# Autodesk Inventor assembly: Zmotionassembly(right)1
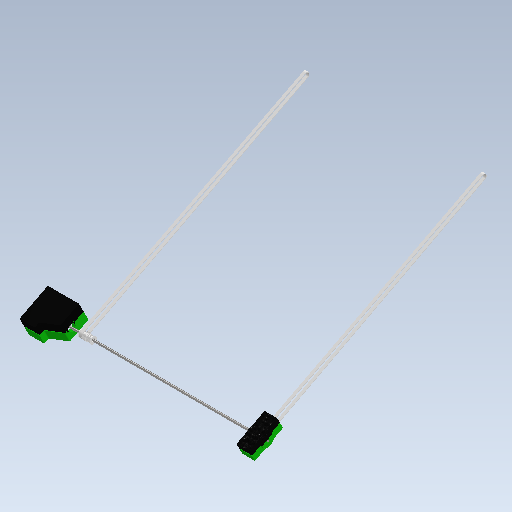
[picture p0: Inventor's stored thumbnail of the model, 512x512]
Saved by Autodesk Inventor 2020.4 (Build 244396000, 396)
## iProperties
Created: 2021-03-29
Part Number: Zmotionassembly(right)1
Document SubType Name: Assembly
Designer: AOB
Mass: 162.106 g
Surface Area: 1029.45 cm^2
Volume: 151.649 cm^3
Density: 1.06896 g/cm^3
Author: AOB
## Documents named in this file (5)
- C:\Users\marti\Documents\Inventor\ProjectBoron\Boron Ultima\Zmotionassembly(right)1.iam
- C:\Users\marti\Documents\Inventor\ProjectBoron\Boron Ultima\Z-powertrain(right)1.iam
- C:\Users\marti\Documents\Inventor\ProjectBoron\Boron Ultima\bottom idler housing(right)1.iam
- C:\Users\marti\Documents\Inventor\ProjectBoron\Boron Ultima\zmotorblock(right)1.iam
- C:\Users\marti\Documents\Inventor\ProjectBoron\Boron Ultima\z-belt(right)1.ipt
## Components (5 placed, 4 different names)
1. Z-powertrain(right)1:1 [sub-assembly] — Flush:1, Mate:2, Flush:2, Mate:3, Rotational:2, Rotational:3
2. bottom idler housing(right)1:1 [sub-assembly] — Flush:1, Mate:2, Angle:1
3. zmotorblock(right)1:1 [sub-assembly] — Flush:2, Mate:3, Angle:2
4. z-belt(right)1:1 — Angle:1, Angle:3, Rotational:2
5. z-belt(right)1:2 — Angle:3, Angle:2, Rotational:3
## Relationships (9: Angle 3, Flush 2, Mate 2, RevoluteJoint 2)
- Flush:1: Z-powertrain(right)1:1 ↔ bottom idler housing(right)1:1
- Mate:2: Z-powertrain(right)1:1 ↔ bottom idler housing(right)1:1
- Flush:2: Z-powertrain(right)1:1 ↔ zmotorblock(right)1:1
- Mate:3: Z-powertrain(right)1:1 ↔ zmotorblock(right)1:1
- Angle:1 (180 deg): bottom idler housing(right)1:1 ↔ z-belt(right)1:1
- Angle:3 (180 deg): z-belt(right)1:1 ↔ z-belt(right)1:2
- Angle:2 (0 deg): zmotorblock(right)1:1 ↔ z-belt(right)1:2
- Rotational:2 [RevoluteJoint] (-0.5 mm): Z-powertrain(right)1:1 ↔ z-belt(right)1:1
- Rotational:3 [RevoluteJoint] (-1.9 mm): Z-powertrain(right)1:1 ↔ z-belt(right)1:2
